# Autodesk Inventor assembly: Forklift.A001
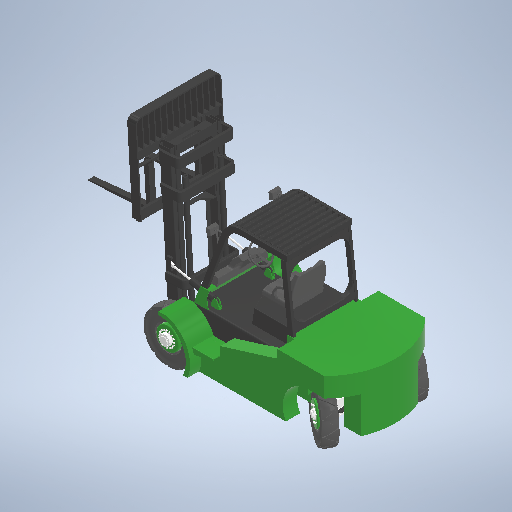
[picture p0: Inventor's stored thumbnail of the model, 512x512]
Saved by Autodesk Inventor 2025.1 (Build 291241000, 241)
## iProperties
Created: 2021-06-18
Part Number: Forklift.A001
Description: STEP AP214
Document SubType Name: Assembly
Designer: victo
Sending System: SolidWorks 2016
Preprocessor: SwSTEP 2.0
Title: Assem2.STEP
Revision Number: ANY
## Documents named in this file (27)
- C:\Users\victo\Downloads\forklift-132.snapshot.1\Forklift.A001\Forklift.A001\Forklift.A001.iam
- C:\Users\victo\Downloads\forklift-132.snapshot.1\Forklift.A001\Forklift.A001\Base back.ipt
- C:\Users\victo\Downloads\forklift-132.snapshot.1\Forklift.A001\Forklift.A001\Base Part.ipt
- C:\Users\victo\Downloads\forklift-132.snapshot.1\Forklift.A001\Forklift.A001\Base side.ipt
- C:\Users\victo\Downloads\forklift-132.snapshot.1\Forklift.A001\Forklift.A001\Base side2.ipt
- C:\Users\victo\Downloads\forklift-132.snapshot.1\Forklift.A001\Forklift.A001\Base back2.ipt
- C:\Users\victo\Downloads\forklift-132.snapshot.1\Forklift.A001\Forklift.A001\Base front.ipt
- C:\Users\victo\Downloads\forklift-132.snapshot.1\Forklift.A001\Forklift.A001\Part9.ipt
- C:\Users\victo\Downloads\forklift-132.snapshot.1\Forklift.A001\Forklift.A001\ceiling.ipt
- C:\Users\victo\Downloads\forklift-132.snapshot.1\Forklift.A001\Forklift.A001\stearing.ipt
- C:\Users\victo\Downloads\forklift-132.snapshot.1\Forklift.A001\Forklift.A001\rear wheel.ipt
- C:\Users\victo\Downloads\forklift-132.snapshot.1\Forklift.A001\Forklift.A001\link.ipt
- C:\Users\victo\Downloads\forklift-132.snapshot.1\Forklift.A001\Forklift.A001\barrel.ipt
- C:\Users\victo\Downloads\forklift-132.snapshot.1\Forklift.A001\Forklift.A001\barrel 2.ipt
- C:\Users\victo\Downloads\forklift-132.snapshot.1\Forklift.A001\Forklift.A001\rod.ipt
- C:\Users\victo\Downloads\forklift-132.snapshot.1\Forklift.A001\Forklift.A001\mast.ipt
- C:\Users\victo\Downloads\forklift-132.snapshot.1\Forklift.A001\Forklift.A001\mast in.ipt
- C:\Users\victo\Downloads\forklift-132.snapshot.1\Forklift.A001\Forklift.A001\FORK SUPPORT.ipt
- C:\Users\victo\Downloads\forklift-132.snapshot.1\Forklift.A001\Forklift.A001\fork.ipt
- C:\Users\victo\Downloads\forklift-132.snapshot.1\Forklift.A001\Forklift.A001\SEAT2.ipt
- C:\Users\victo\Downloads\forklift-132.snapshot.1\Forklift.A001\Forklift.A001\SEAT.ipt
- C:\Users\victo\Downloads\forklift-132.snapshot.1\Forklift.A001\Forklift.A001\Part7.ipt
- C:\Users\victo\Downloads\forklift-132.snapshot.1\Forklift.A001\Forklift.A001\LIGHT.ipt
- C:\Users\victo\Downloads\forklift-132.snapshot.1\Forklift.A001\Forklift.A001\front wheel.ipt
- C:\Users\victo\Downloads\forklift-132.snapshot.1\Forklift.A001\Forklift.A001\rear wheel2.ipt
- C:\Users\victo\Downloads\forklift-132.snapshot.1\Forklift.A001\Forklift.A001\Part8.ipt
- C:\Users\victo\Downloads\forklift-132.snapshot.1\Forklift.A001\Forklift.A001\Part10.ipt
## Components (36 placed, 35 different names)
1. Base back_1 — Flush:1, Mate:43
2. Base Part_2
3. Base side_3
4. Base side2_4
5. Base back2_5 — Mate:28, Mate:29, Mate:30, Mate:33, Mate:34, Flush:1, Mate:43
6. Base front_6
7. Part9_7 — Mate:4, Mate:5, Mate:9, Mate:10, Rotational:1
8. ceiling_8
9. stearing_9 — Mate:28, Mate:32, Mate:36
10. rear wheel_10 — Mate:29, Mate:30, Mate:31, Mate:40, Mate:41, Mate:42, Rotation:1
11. rear wheel_11 — Mate:33, Mate:34, Mate:35, Mate:37, Mate:38, Mate:39
12. link_12 — Mate:31, Mate:32
13. link_13 — Mate:35, Mate:36
14. barrel_14 — Mate:14, Mate:15
15. barrel_15 — Mate:18, Mate:19
16. barrel 2_16 — Mate:14, Mate:15, Mate:16
17. barrel 2_17 — Mate:18, Mate:19, Mate:20
18. rod_18 — Mate:16, Mate:17
19. rod_19 — Mate:20, Mate:21
20. mast_20 — Mate:17, Mate:21, Rotational:1, Slider:1
21. mast in_21 — Slider:1, Mate:23, Slider:2
22. FORK SUPPORT_22 — Mate:23, Slider:2, Mate:24, Mate:25, Angle:1, Angle:2, Mate:26, Mate:27
23. fork_23 — Mate:24, Angle:2, Mate:26
24. fork_24 — Mate:25, Angle:1, Mate:27
25. SEAT2_25
26. SEAT_26
27. Part7_27 — Mate:2, Mate:3
28. LIGHT_28
29. LIGHT_29
30. front wheel_30 — Mate:6, Mate:7, Mate:8
31. rear wheel2_31 — Mate:40, Mate:41, Mate:42
32. rear wheel2_32 — Mate:37, Mate:38, Mate:39
33. front wheel_33 — Mate:11, Mate:12, Mate:13
34. Part8:1 — Mate:2, Mate:3, Rotation:1
35. Part10:1 — Mate:4, Mate:5, Mate:6, Mate:7, Mate:8
36. Part10:2 — Mate:9, Mate:10, Mate:11, Mate:12, Mate:13
## Relationships (48: Mate 41, TranslationJoint 2, Angle 2, RevoluteJoint 1, RelateRotation 1, Flush 1)
- Mate:2: Part7_27 ↔ Part8:1
- Mate:3: Part7_27 ↔ Part8:1
- Mate:4: Part9_7 ↔ Part10:1
- Mate:5: Part9_7 ↔ Part10:1
- Mate:6: front wheel_30 ↔ Part10:1
- Mate:7: front wheel_30 ↔ Part10:1
- Mate:8: front wheel_30 ↔ Part10:1
- Mate:9: Part9_7 ↔ Part10:2
- Mate:10: Part9_7 ↔ Part10:2
- Mate:11: front wheel_33 ↔ Part10:2
- Mate:12: front wheel_33 ↔ Part10:2
- Mate:13: front wheel_33 ↔ Part10:2
- Mate:14: barrel_14 ↔ barrel 2_16
- Mate:15 (2.5 mm): barrel_14 ↔ barrel 2_16
- Mate:16: barrel 2_16 ↔ rod_18
- Mate:17: rod_18 ↔ mast_20
- Mate:18: barrel_15 ↔ barrel 2_17
- Mate:19 (2.5 mm): barrel_15 ↔ barrel 2_17
- Mate:20: barrel 2_17 ↔ rod_19
- Mate:21: rod_19 ↔ mast_20
- Rotational:1 [RevoluteJoint]: Part9_7 ↔ mast_20
- Slider:1 [TranslationJoint] (70 mm): mast_20 ↔ mast in_21
- Mate:23: mast in_21 ↔ FORK SUPPORT_22
- Slider:2 [TranslationJoint]: mast in_21 ↔ FORK SUPPORT_22
- Mate:24: FORK SUPPORT_22 ↔ fork_23
- Mate:25: FORK SUPPORT_22 ↔ fork_24
- Angle:1 (0 deg): FORK SUPPORT_22 ↔ fork_24
- Angle:2 (0 deg): FORK SUPPORT_22 ↔ fork_23
- Mate:26 (250 mm): FORK SUPPORT_22 ↔ fork_23
- Mate:27 (250 mm): FORK SUPPORT_22 ↔ fork_24
- Mate:28: Base back2_5 ↔ stearing_9
- Mate:29: Base back2_5 ↔ rear wheel_10
- Mate:30: Base back2_5 ↔ rear wheel_10
- Mate:31: rear wheel_10 ↔ link_12
- Mate:32: stearing_9 ↔ link_12
- Mate:33: Base back2_5 ↔ rear wheel_11
- Mate:34: Base back2_5 ↔ rear wheel_11
- Mate:35: rear wheel_11 ↔ link_13
- Mate:36: stearing_9 ↔ link_13
- Mate:37: rear wheel_11 ↔ rear wheel2_32
- Mate:38: rear wheel_11 ↔ rear wheel2_32
- Mate:39: rear wheel_11 ↔ rear wheel2_32
- Mate:40: rear wheel_10 ↔ rear wheel2_31
- Mate:41: rear wheel_10 ↔ rear wheel2_31
- Mate:42: rear wheel_10 ↔ rear wheel2_31
- Rotation:1 [RelateRotation] (0.395 ul): rear wheel_10 ↔ Part8:1
- Flush:1 (22.11 mm): Base back_1 ↔ Base back2_5
- Mate:43 (250 mm): Base back_1 ↔ Base back2_5
